# Autodesk Inventor assembly: CycloidalGearBoxV3_Assembly
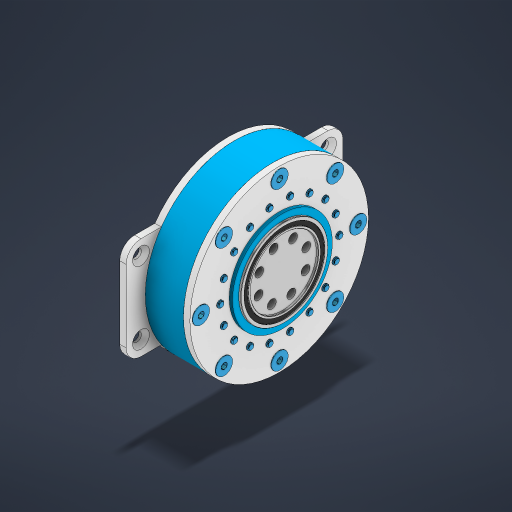
[picture p0: Inventor's stored thumbnail of the model, 512x512]
Saved by Autodesk Inventor 2024 (Build 280153000, 153)
## iProperties
Created: 2024-03-23
Part Number: CycloidalGearBoxV3_Assembly
Document SubType Name: Assembly
Designer: avsar
Author: avsar
## Documents named in this file (21)
- C:\Users\avsar\Documents\Inventor\RCR_Arm\Arm_V4\CycloidalGearBoxes\CycloidalGearboxV3\CycloidalGearBoxV3_Assembly.iam
- C:\Users\avsar\Documents\Inventor\RCR_Arm\Arm_V4\CycloidalGearBoxes\StageOneGearBox\HousingFaceInput.ipt
- C:\Users\avsar\Documents\Inventor\RCR_Arm\COTS\ISO Standard Hardware\Screws\Sockethead Screws\Countersunk Screws\M3 x 0.5mm\(M3 x 0.5 x 25) Sockethead Countersunk Screw.ipt
- C:\Users\avsar\Documents\Inventor\RCR_Arm\COTS\Motion\Bearings\Flanged Bearings\10x15x4mm Flanged Bearing.ipt
- C:\Users\avsar\Documents\Inventor\RCR_Arm\COTS\Motion\Bearings\Thrust Bearings\3mm ID x 8mm OD Thrust Ball Bearing.ipt
- C:\Users\avsar\Documents\Inventor\RCR_Arm\Arm_V4\CycloidalGearBoxes\CycloidalGearboxV3\RollerSpacers\ThrustRollerSpacer.ipt
- C:\Users\avsar\Documents\Inventor\RCR_Arm\Arm_V4\CycloidalGearBoxes\CycloidalGearboxV3\EccentricShaftSpacer.ipt
- C:\Users\avsar\Documents\Inventor\RCR_Arm\Arm_V4\CycloidalGearBoxes\CycloidalGearboxV3\CycloidalDisk.ipt
- C:\Users\avsar\Documents\Inventor\RCR_Arm\Arm_V4\CycloidalGearBoxes\CycloidalGearboxV3\EccentricShaft.ipt
- C:\Users\avsar\Documents\Inventor\RCR_Arm\COTS\Motion\Bearings\Standard Bearings\16mm ID x 22mm OD x 4mm Thickness Ball Bearing.ipt
- C:\Users\avsar\Documents\Inventor\RCR_Arm\COTS\ISO Standard Hardware\Screws\Sockethead Screws\Buttonhead Screws\M3 x 0.5mm\(M3 x 0.5 x 16) Sockethead Buttonhead Screw.ipt
- C:\Users\avsar\Documents\Inventor\RCR_Arm\Arm_V4\CycloidalGearBoxes\CycloidalGearboxV3\InnerBearingButtonheadShims.ipt
- C:\Users\avsar\Documents\Inventor\RCR_Arm\Arm_V4\CycloidalGearBoxes\CycloidalGearboxV3\InnerPins\InnerPinOutputSpacer.ipt
- C:\Users\avsar\Documents\Inventor\RCR_Arm\Arm_V4\CycloidalGearBoxes\CycloidalGearboxV3\OutPutPlate.ipt
- C:\Users\avsar\Documents\Inventor\RCR_Arm\Arm_V4\CycloidalGearBoxes\CycloidalGearboxV3\RollerSpacers\3mm ID x 4mm OD x 2mm Length Spacer.ipt
- C:\Users\avsar\Documents\Inventor\RCR_Arm\Arm_V4\CycloidalGearBoxes\CycloidalGearboxV3\RollerSpacers\StandardRollerSpacer.ipt
- C:\Users\avsar\Documents\Inventor\RCR_Arm\Arm_V4\CycloidalGearBoxes\CycloidalGearboxV3\HousingLid.ipt
- C:\Users\avsar\Documents\Inventor\RCR_Arm\Arm_V4\CycloidalGearBoxes\CycloidalGearboxV3\Gearbox_MainBody.ipt
- C:\Users\avsar\Documents\Inventor\RCR_Arm\COTS\goBilda\Motion\Bearings\32mm ID Flanged Ball Bearing (39mm OD, 5mm Thickness).ipt
- C:\Users\avsar\Documents\Inventor\RCR_Arm\Arm_V4\CycloidalGearBoxes\CycloidalGearboxV3\OutputBearingDistanceRing.ipt
- C:\Users\avsar\Documents\Inventor\RCR_Arm\COTS\ISO Standard Hardware\Screws\Sockethead Screws\Countersunk Screws\M4 x 0.7mm\(M4 x 0.7 x 10) Sockethead Countersunk Screw.ipt
## Components (107 placed, 20 different names)
1. HousingFaceInput:1 — Mate:1, Mate:2, Flush:1, Mate:3, Flush:2, Mate:4, Flush:3, Mate:5, Flush:4, Mate:6, Flush:5, Mate:7, Flush:6, Mate:8, Flush:7, Mate:9, Flush:8, Mate:10, Flush:9, Mate:11, Flush:10, Mate:12, Flush:11, Mate:13, Flush:12, Mate:14, Flush:13, Flush:14, Mate:15, Mate:16, Flush:15, Mate:17, Flush:16, Mate:18, Flush:17, Mate:19, Mate:20, Mate:21, Mate:26, Mate:91, Mate:97, Mate:103, Mate:109, Mate:115, Mate:129, Mate:131, Mate:133, Mate:135, Mate:137, Mate:139, Mate:141, Mate:143, Mate:145, Mate:147, Mate:149, Mate:151, Mate:154, Mate:155, Mate:156, Flush:20, Mate:163, Flush:21, Mate:164, Flush:22, Mate:165, Flush:23, Mate:166, Flush:24, Mate:167, Flush:25, Mate:168, Flush:26, Mate:169, Flush:27, Mate:170
2. 10x15x4mm Flanged Bearing:1 — Mate:20, Mate:21, Mate:30, Mate:31
3. EccentricShaftSpacer:1 — Mate:30, Mate:31, Mate:32, Mate:33
4. CycloidalDisk:1 — Flush:18, Mate:34, Mate:46, Tangent:1, Mate:51, Tangent:3, Mate:56, Tangent:5, Mate:69, Tangent:7, Mate:70, Tangent:9, Mate:71, Tangent:11, Tangent:13
5. EccentricShaft:1 — Mate:32, Mate:33, Mate:35, Mate:36, Mate:38, Mate:39
6. 16mm ID x 22mm OD x 4mm Thickness Ball Bearing:1 — Flush:18, Mate:34, Mate:35, Mate:36
7. CycloidalDisk:2 — Tangent:2, Tangent:4, Tangent:6, Tangent:8, Tangent:10, Tangent:12
8. OutPutPlate:1 — Mate:84, Mate:85, Mate:86
9. 16mm ID x 22mm OD x 4mm Thickness Ball Bearing:2 — Mate:38, Mate:39
10. StandardRollerSpacer:1 — Mate:129, Mate:130
11. StandardRollerSpacer:2 — Mate:131, Mate:132
12. StandardRollerSpacer:3 — Mate:133, Mate:134
13. StandardRollerSpacer:4 — Mate:135, Mate:136, Mate:153
14. StandardRollerSpacer:5 — Mate:137, Mate:138
15. StandardRollerSpacer:6 — Mate:139, Mate:140
16. StandardRollerSpacer:7 — Mate:141, Mate:142
17. StandardRollerSpacer:8 — Mate:143, Mate:144
18. StandardRollerSpacer:9 — Mate:145, Mate:146
19. StandardRollerSpacer:10 — Mate:147, Mate:148
20. StandardRollerSpacer:11 — Mate:149, Mate:150
21. StandardRollerSpacer:12 — Mate:151, Mate:152
22. HousingLid:1 — Mate:153, Mate:157, Mate:158, Mate:161, Mate:162, Flush:28, Mate:171, Flush:29, Mate:172, Flush:30, Mate:173, Flush:31, Mate:174, Flush:32, Mate:175, Flush:33, Mate:176, Flush:34, Mate:177, Flush:35, Mate:178
23. Gearbox_MainBody:1 — Mate:154, Mate:155, Mate:156, Mate:157, Mate:158
24. 32mm ID Flanged Ball Bearing (39mm OD, 5mm Thickness):1 — Mate:159, Mate:160, Mate:162
25. OutputBearingDistanceRing:1 — Mate:159, Mate:160, Mate:161
26. (M4 x 0.7 x 10) Sockethead Countersunk Screw:1 — Flush:20, Mate:163
27. (M4 x 0.7 x 10) Sockethead Countersunk Screw:2 — Flush:21, Mate:164
28. (M4 x 0.7 x 10) Sockethead Countersunk Screw:3 — Flush:22, Mate:165
29. (M4 x 0.7 x 10) Sockethead Countersunk Screw:4 — Flush:23, Mate:166
30. (M4 x 0.7 x 10) Sockethead Countersunk Screw:5 — Flush:24, Mate:167
31. (M4 x 0.7 x 10) Sockethead Countersunk Screw:6 — Flush:25, Mate:168
32. (M4 x 0.7 x 10) Sockethead Countersunk Screw:7 — Flush:26, Mate:169
33. (M4 x 0.7 x 10) Sockethead Countersunk Screw:8 — Flush:27, Mate:170
34. (M4 x 0.7 x 10) Sockethead Countersunk Screw:9 — Flush:28, Mate:171
35. (M4 x 0.7 x 10) Sockethead Countersunk Screw:10 — Flush:29, Mate:172
36. (M4 x 0.7 x 10) Sockethead Countersunk Screw:11 — Flush:30, Mate:173
37. (M4 x 0.7 x 10) Sockethead Countersunk Screw:12 — Flush:31, Mate:174
38. (M4 x 0.7 x 10) Sockethead Countersunk Screw:13 — Flush:32, Mate:175
39. (M4 x 0.7 x 10) Sockethead Countersunk Screw:14 — Flush:33, Mate:176
40. (M4 x 0.7 x 10) Sockethead Countersunk Screw:15 — Flush:34, Mate:177
41. (M4 x 0.7 x 10) Sockethead Countersunk Screw:16 — Flush:35, Mate:178
42. (M3 x 0.5 x 25) Sockethead Countersunk Screw:12 — Flush:11, Mate:13, Mate:98, Mate:126
43. (M3 x 0.5 x 25) Sockethead Countersunk Screw:13 — Flush:12, Mate:14, Mate:140
44. (M3 x 0.5 x 25) Sockethead Countersunk Screw:14 — Flush:13, Mate:15, Mate:138
45. (M3 x 0.5 x 25) Sockethead Countersunk Screw:15 — Flush:14, Mate:16, Mate:92, Mate:128
46. (M3 x 0.5 x 25) Sockethead Countersunk Screw:16 — Flush:15, Mate:17, Mate:136
47. (M3 x 0.5 x 25) Sockethead Countersunk Screw:17 — Flush:16, Mate:18, Mate:134
48. (M3 x 0.5 x 25) Sockethead Countersunk Screw:18 — Flush:17, Mate:19, Mate:25, Mate:28
49. (M3 x 0.5 x 25) Sockethead Countersunk Screw:1 — Mate:1, Mate:2, Mate:130
50. (M3 x 0.5 x 25) Sockethead Countersunk Screw:2 — Flush:1, Mate:3, Mate:132
51. (M3 x 0.5 x 25) Sockethead Countersunk Screw:3 — Flush:2, Mate:4, Mate:116, Mate:120
52. (M3 x 0.5 x 25) Sockethead Countersunk Screw:4 — Flush:3, Mate:5, Mate:152
53. (M3 x 0.5 x 25) Sockethead Countersunk Screw:5 — Flush:4, Mate:6, Mate:150
54. (M3 x 0.5 x 25) Sockethead Countersunk Screw:6 — Flush:5, Mate:7, Mate:110, Mate:122
55. (M3 x 0.5 x 25) Sockethead Countersunk Screw:7 — Flush:6, Mate:8, Mate:148
56. (M3 x 0.5 x 25) Sockethead Countersunk Screw:8 — Flush:7, Mate:9, Mate:146
57. (M3 x 0.5 x 25) Sockethead Countersunk Screw:9 — Flush:8, Mate:10, Mate:104, Mate:124
58. (M3 x 0.5 x 25) Sockethead Countersunk Screw:10 — Flush:9, Mate:11, Mate:144
59. (M3 x 0.5 x 25) Sockethead Countersunk Screw:11 — Flush:10, Mate:12, Mate:142
60. (M3 x 0.5 x 16) Sockethead Buttonhead Screw:1 — Mate:42, Mate:43, Mate:79
61. InnerBearingButtonheadShims:1 — Mate:42, Mate:43, Mate:44, Mate:45, Mate:46
62. ThrustRollerSpacer:2 — Mate:44, Mate:45, Tangent:1, Tangent:2, Mate:78
63. (M3 x 0.5 x 16) Sockethead Buttonhead Screw:2 — Mate:77
64. InnerBearingButtonheadShims:2 — Mate:51
65. ThrustRollerSpacer:3 — Tangent:3, Tangent:4, Mate:76
66. (M3 x 0.5 x 16) Sockethead Buttonhead Screw:3 — Mate:81, Mate:86
67. InnerBearingButtonheadShims:3 — Mate:56
68. ThrustRollerSpacer:4 — Tangent:5, Tangent:6, Mate:80
69. (M3 x 0.5 x 16) Sockethead Buttonhead Screw:4 — Mate:83
70. InnerBearingButtonheadShims:4 — Mate:69
71. ThrustRollerSpacer:5 — Tangent:7, Tangent:8, Mate:82
72. (M3 x 0.5 x 16) Sockethead Buttonhead Screw:5 — Mate:73
73. InnerBearingButtonheadShims:5 — Mate:70
74. ThrustRollerSpacer:6 — Tangent:9, Tangent:10, Mate:72
75. (M3 x 0.5 x 16) Sockethead Buttonhead Screw:6 — Mate:75, Mate:85
76. InnerBearingButtonheadShims:6 — Mate:71
77. ThrustRollerSpacer:7 — Tangent:11, Tangent:12, Mate:74
78. InnerPinOutputSpacer:1 — Mate:72, Mate:73
79. InnerPinOutputSpacer:2 — Mate:74, Mate:75, Mate:84
80. InnerPinOutputSpacer:3 — Mate:76, Mate:77
81. InnerPinOutputSpacer:4 — Mate:78, Mate:79
82. InnerPinOutputSpacer:5 — Mate:80, Mate:81
83. InnerPinOutputSpacer:6 — Mate:82, Mate:83
84. 3mm ID x 8mm OD Thrust Ball Bearing:5 — Mate:125
85. 3mm ID x 8mm OD Thrust Ball Bearing:6 — Mate:97
86. ThrustRollerSpacer:9 — Mate:98
87. 3mm ID x 8mm OD Thrust Ball Bearing:7 — Mate:123
88. 3mm ID x 8mm OD Thrust Ball Bearing:8 — Mate:103
89. ThrustRollerSpacer:10 — Mate:104
90. 3mm ID x 8mm OD Thrust Ball Bearing:9 — Mate:121
91. 3mm ID x 8mm OD Thrust Ball Bearing:10 — Mate:109
92. ThrustRollerSpacer:11 — Mate:110
93. 3mm ID x 8mm OD Thrust Ball Bearing:11 — Mate:119
94. 3mm ID x 8mm OD Thrust Ball Bearing:12 — Mate:115
95. ThrustRollerSpacer:12 — Mate:116
96. 3mm ID x 4mm OD x 2mm Length Spacer:1 — Mate:117, Mate:118
97. 3mm ID x 4mm OD x 2mm Length Spacer:2 — Mate:123, Mate:124
98. 3mm ID x 4mm OD x 2mm Length Spacer:3 — Mate:125, Mate:126
99. 3mm ID x 4mm OD x 2mm Length Spacer:4 — Mate:127, Mate:128
100. 3mm ID x 4mm OD x 2mm Length Spacer:5 — Mate:121, Mate:122
101. 3mm ID x 4mm OD x 2mm Length Spacer:6 — Mate:119, Mate:120
102. 3mm ID x 8mm OD Thrust Ball Bearing:3 — Mate:127
103. 3mm ID x 8mm OD Thrust Ball Bearing:4 — Mate:91
104. ThrustRollerSpacer:8 — Mate:92
105. 3mm ID x 8mm OD Thrust Ball Bearing:1 — Mate:25, Mate:26, Mate:27, Mate:29
106. 3mm ID x 8mm OD Thrust Ball Bearing:2 — Mate:40, Mate:41, Mate:117
107. ThrustRollerSpacer:1 — Mate:27, Mate:28, Mate:29, Mate:40, Mate:41, Tangent:13, Mate:118
## Relationships (223: Mate 175, Flush 35, Tangent 13)
- Mate:1: HousingFaceInput:1 ↔ (M3 x 0.5 x 25) Sockethead Countersunk Screw:1
- Mate:2: HousingFaceInput:1 ↔ (M3 x 0.5 x 25) Sockethead Countersunk Screw:1
- Flush:1 (-0.085 mm): HousingFaceInput:1 ↔ (M3 x 0.5 x 25) Sockethead Countersunk Screw:2
- Mate:3: HousingFaceInput:1 ↔ (M3 x 0.5 x 25) Sockethead Countersunk Screw:2
- Flush:2 (-0.085 mm): HousingFaceInput:1 ↔ (M3 x 0.5 x 25) Sockethead Countersunk Screw:3
- Mate:4: HousingFaceInput:1 ↔ (M3 x 0.5 x 25) Sockethead Countersunk Screw:3
- Flush:3 (-0.085 mm): HousingFaceInput:1 ↔ (M3 x 0.5 x 25) Sockethead Countersunk Screw:4
- Mate:5: HousingFaceInput:1 ↔ (M3 x 0.5 x 25) Sockethead Countersunk Screw:4
- Flush:4 (-0.085 mm): HousingFaceInput:1 ↔ (M3 x 0.5 x 25) Sockethead Countersunk Screw:5
- Mate:6: HousingFaceInput:1 ↔ (M3 x 0.5 x 25) Sockethead Countersunk Screw:5
- Flush:5 (-0.085 mm): HousingFaceInput:1 ↔ (M3 x 0.5 x 25) Sockethead Countersunk Screw:6
- Mate:7: HousingFaceInput:1 ↔ (M3 x 0.5 x 25) Sockethead Countersunk Screw:6
- Flush:6 (-0.085 mm): HousingFaceInput:1 ↔ (M3 x 0.5 x 25) Sockethead Countersunk Screw:7
- Mate:8: HousingFaceInput:1 ↔ (M3 x 0.5 x 25) Sockethead Countersunk Screw:7
- Flush:7 (-0.085 mm): HousingFaceInput:1 ↔ (M3 x 0.5 x 25) Sockethead Countersunk Screw:8
- Mate:9: HousingFaceInput:1 ↔ (M3 x 0.5 x 25) Sockethead Countersunk Screw:8
- Flush:8 (-0.085 mm): HousingFaceInput:1 ↔ (M3 x 0.5 x 25) Sockethead Countersunk Screw:9
- Mate:10: HousingFaceInput:1 ↔ (M3 x 0.5 x 25) Sockethead Countersunk Screw:9
- Flush:9 (-0.085 mm): HousingFaceInput:1 ↔ (M3 x 0.5 x 25) Sockethead Countersunk Screw:10
- Mate:11: HousingFaceInput:1 ↔ (M3 x 0.5 x 25) Sockethead Countersunk Screw:10
- Flush:10 (-0.085 mm): HousingFaceInput:1 ↔ (M3 x 0.5 x 25) Sockethead Countersunk Screw:11
- Mate:12: HousingFaceInput:1 ↔ (M3 x 0.5 x 25) Sockethead Countersunk Screw:11
- Flush:11 (-0.085 mm): HousingFaceInput:1 ↔ (M3 x 0.5 x 25) Sockethead Countersunk Screw:12
- Mate:13: HousingFaceInput:1 ↔ (M3 x 0.5 x 25) Sockethead Countersunk Screw:12
- Flush:12 (-0.085 mm): HousingFaceInput:1 ↔ (M3 x 0.5 x 25) Sockethead Countersunk Screw:13
- Mate:14: HousingFaceInput:1 ↔ (M3 x 0.5 x 25) Sockethead Countersunk Screw:13
- Flush:13 (-0.085 mm): HousingFaceInput:1 ↔ (M3 x 0.5 x 25) Sockethead Countersunk Screw:14
- Flush:14 (-0.085 mm): HousingFaceInput:1 ↔ (M3 x 0.5 x 25) Sockethead Countersunk Screw:15
- Mate:15: HousingFaceInput:1 ↔ (M3 x 0.5 x 25) Sockethead Countersunk Screw:14
- Mate:16: HousingFaceInput:1 ↔ (M3 x 0.5 x 25) Sockethead Countersunk Screw:15
- Flush:15 (-0.085 mm): HousingFaceInput:1 ↔ (M3 x 0.5 x 25) Sockethead Countersunk Screw:16
- Mate:17: HousingFaceInput:1 ↔ (M3 x 0.5 x 25) Sockethead Countersunk Screw:16
- Flush:16 (-0.085 mm): HousingFaceInput:1 ↔ (M3 x 0.5 x 25) Sockethead Countersunk Screw:17
- Mate:18: HousingFaceInput:1 ↔ (M3 x 0.5 x 25) Sockethead Countersunk Screw:17
- Flush:17 (-0.085 mm): HousingFaceInput:1 ↔ (M3 x 0.5 x 25) Sockethead Countersunk Screw:18
- Mate:19: HousingFaceInput:1 ↔ (M3 x 0.5 x 25) Sockethead Countersunk Screw:18
- Mate:20: HousingFaceInput:1 ↔ 10x15x4mm Flanged Bearing:1
- Mate:21: HousingFaceInput:1 ↔ 10x15x4mm Flanged Bearing:1
- Mate:25: (M3 x 0.5 x 25) Sockethead Countersunk Screw:18 ↔ 3mm ID x 8mm OD Thrust Ball Bearing:1
- Mate:26: HousingFaceInput:1 ↔ 3mm ID x 8mm OD Thrust Ball Bearing:1
- Mate:27: 3mm ID x 8mm OD Thrust Ball Bearing:1 ↔ ThrustRollerSpacer:1
- Mate:28: (M3 x 0.5 x 25) Sockethead Countersunk Screw:18 ↔ ThrustRollerSpacer:1
- Mate:29: 3mm ID x 8mm OD Thrust Ball Bearing:1 ↔ ThrustRollerSpacer:1
- Mate:30: 10x15x4mm Flanged Bearing:1 ↔ EccentricShaftSpacer:1
- Mate:31: 10x15x4mm Flanged Bearing:1 ↔ EccentricShaftSpacer:1
- Mate:32: EccentricShaftSpacer:1 ↔ EccentricShaft:1
- Mate:33: EccentricShaftSpacer:1 ↔ EccentricShaft:1
- Flush:18: CycloidalDisk:1 ↔ 16mm ID x 22mm OD x 4mm Thickness Ball Bearing:1
- Mate:34: CycloidalDisk:1 ↔ 16mm ID x 22mm OD x 4mm Thickness Ball Bearing:1
- Mate:35: EccentricShaft:1 ↔ 16mm ID x 22mm OD x 4mm Thickness Ball Bearing:1
- Mate:36: EccentricShaft:1 ↔ 16mm ID x 22mm OD x 4mm Thickness Ball Bearing:1
- [Flush]: CycloidalDisk:2 ↔ 16mm ID x 22mm OD x 4mm Thickness Ball Bearing:2
- [Mate]: CycloidalDisk:2 ↔ 16mm ID x 22mm OD x 4mm Thickness Ball Bearing:2
- Mate:38: EccentricShaft:1 ↔ 16mm ID x 22mm OD x 4mm Thickness Ball Bearing:2
- Mate:39: EccentricShaft:1 ↔ 16mm ID x 22mm OD x 4mm Thickness Ball Bearing:2
- Mate:40: 3mm ID x 8mm OD Thrust Ball Bearing:2 ↔ ThrustRollerSpacer:1
- Mate:41: 3mm ID x 8mm OD Thrust Ball Bearing:2 ↔ ThrustRollerSpacer:1
- Mate:42: (M3 x 0.5 x 16) Sockethead Buttonhead Screw:1 ↔ InnerBearingButtonheadShims:1
- Mate:43: (M3 x 0.5 x 16) Sockethead Buttonhead Screw:1 ↔ InnerBearingButtonheadShims:1
- Mate:44: InnerBearingButtonheadShims:1 ↔ ThrustRollerSpacer:2
- Mate:45: InnerBearingButtonheadShims:1 ↔ ThrustRollerSpacer:2
- Mate:46: CycloidalDisk:1 ↔ InnerBearingButtonheadShims:1
- Tangent:1: CycloidalDisk:1 ↔ ThrustRollerSpacer:2
- Tangent:2: CycloidalDisk:2 ↔ ThrustRollerSpacer:2
- [Mate]: (M3 x 0.5 x 16) Sockethead Buttonhead Screw:2 ↔ InnerBearingButtonheadShims:2
- [Mate]: (M3 x 0.5 x 16) Sockethead Buttonhead Screw:2 ↔ InnerBearingButtonheadShims:2
- [Mate]: InnerBearingButtonheadShims:2 ↔ ThrustRollerSpacer:3
- [Mate]: InnerBearingButtonheadShims:2 ↔ ThrustRollerSpacer:3
- Mate:51: CycloidalDisk:1 ↔ InnerBearingButtonheadShims:2
- Tangent:3: CycloidalDisk:1 ↔ ThrustRollerSpacer:3
- Tangent:4: CycloidalDisk:2 ↔ ThrustRollerSpacer:3
- [Mate]: (M3 x 0.5 x 16) Sockethead Buttonhead Screw:3 ↔ InnerBearingButtonheadShims:3
- [Mate]: (M3 x 0.5 x 16) Sockethead Buttonhead Screw:3 ↔ InnerBearingButtonheadShims:3
- [Mate]: InnerBearingButtonheadShims:3 ↔ ThrustRollerSpacer:4
- [Mate]: InnerBearingButtonheadShims:3 ↔ ThrustRollerSpacer:4
- Mate:56: CycloidalDisk:1 ↔ InnerBearingButtonheadShims:3
- Tangent:5: CycloidalDisk:1 ↔ ThrustRollerSpacer:4
- Tangent:6: CycloidalDisk:2 ↔ ThrustRollerSpacer:4
- [Mate]: (M3 x 0.5 x 16) Sockethead Buttonhead Screw:4 ↔ InnerBearingButtonheadShims:4
- [Mate]: (M3 x 0.5 x 16) Sockethead Buttonhead Screw:4 ↔ InnerBearingButtonheadShims:4
- [Mate]: InnerBearingButtonheadShims:4 ↔ ThrustRollerSpacer:5
- [Mate]: InnerBearingButtonheadShims:4 ↔ ThrustRollerSpacer:5
- [Mate]: (M3 x 0.5 x 16) Sockethead Buttonhead Screw:5 ↔ InnerBearingButtonheadShims:5
- [Mate]: (M3 x 0.5 x 16) Sockethead Buttonhead Screw:5 ↔ InnerBearingButtonheadShims:5
- [Mate]: InnerBearingButtonheadShims:5 ↔ ThrustRollerSpacer:6
- [Mate]: InnerBearingButtonheadShims:5 ↔ ThrustRollerSpacer:6
- [Mate]: (M3 x 0.5 x 16) Sockethead Buttonhead Screw:6 ↔ InnerBearingButtonheadShims:6
- [Mate]: (M3 x 0.5 x 16) Sockethead Buttonhead Screw:6 ↔ InnerBearingButtonheadShims:6
- [Mate]: InnerBearingButtonheadShims:6 ↔ ThrustRollerSpacer:7
- [Mate]: InnerBearingButtonheadShims:6 ↔ ThrustRollerSpacer:7
- Mate:69: CycloidalDisk:1 ↔ InnerBearingButtonheadShims:4
- Tangent:7: CycloidalDisk:1 ↔ ThrustRollerSpacer:5
- Tangent:8: CycloidalDisk:2 ↔ ThrustRollerSpacer:5
- Mate:70: CycloidalDisk:1 ↔ InnerBearingButtonheadShims:5
- Tangent:9: CycloidalDisk:1 ↔ ThrustRollerSpacer:6
- Tangent:10: CycloidalDisk:2 ↔ ThrustRollerSpacer:6
- Mate:71: CycloidalDisk:1 ↔ InnerBearingButtonheadShims:6
- Tangent:11: CycloidalDisk:1 ↔ ThrustRollerSpacer:7
- Tangent:12: CycloidalDisk:2 ↔ ThrustRollerSpacer:7
- Mate:72: ThrustRollerSpacer:6 ↔ InnerPinOutputSpacer:1
- Mate:73: (M3 x 0.5 x 16) Sockethead Buttonhead Screw:5 ↔ InnerPinOutputSpacer:1
- Mate:74: ThrustRollerSpacer:7 ↔ InnerPinOutputSpacer:2
- Mate:75: (M3 x 0.5 x 16) Sockethead Buttonhead Screw:6 ↔ InnerPinOutputSpacer:2
- Mate:76: ThrustRollerSpacer:3 ↔ InnerPinOutputSpacer:3
- Mate:77: (M3 x 0.5 x 16) Sockethead Buttonhead Screw:2 ↔ InnerPinOutputSpacer:3
- Mate:78: ThrustRollerSpacer:2 ↔ InnerPinOutputSpacer:4
- Mate:79: (M3 x 0.5 x 16) Sockethead Buttonhead Screw:1 ↔ InnerPinOutputSpacer:4
- Mate:80: ThrustRollerSpacer:4 ↔ InnerPinOutputSpacer:5
- Mate:81: (M3 x 0.5 x 16) Sockethead Buttonhead Screw:3 ↔ InnerPinOutputSpacer:5
- Mate:82: ThrustRollerSpacer:5 ↔ InnerPinOutputSpacer:6
- Mate:83: (M3 x 0.5 x 16) Sockethead Buttonhead Screw:4 ↔ InnerPinOutputSpacer:6
- Mate:84: OutPutPlate:1 ↔ InnerPinOutputSpacer:2
- Mate:85: OutPutPlate:1 ↔ (M3 x 0.5 x 16) Sockethead Buttonhead Screw:6
- Mate:86: OutPutPlate:1 ↔ (M3 x 0.5 x 16) Sockethead Buttonhead Screw:3
- Tangent:13: CycloidalDisk:1 ↔ ThrustRollerSpacer:1
- [Mate]: 3mm ID x 8mm OD Thrust Ball Bearing:3 ↔ ThrustRollerSpacer:8
- [Mate]: 3mm ID x 8mm OD Thrust Ball Bearing:3 ↔ ThrustRollerSpacer:8
- [Mate]: 3mm ID x 8mm OD Thrust Ball Bearing:4 ↔ ThrustRollerSpacer:8
- [Mate]: 3mm ID x 8mm OD Thrust Ball Bearing:4 ↔ ThrustRollerSpacer:8
- Mate:91: HousingFaceInput:1 ↔ 3mm ID x 8mm OD Thrust Ball Bearing:4
- Mate:92: (M3 x 0.5 x 25) Sockethead Countersunk Screw:15 ↔ ThrustRollerSpacer:8
- [Mate]: 3mm ID x 8mm OD Thrust Ball Bearing:5 ↔ ThrustRollerSpacer:9
- [Mate]: 3mm ID x 8mm OD Thrust Ball Bearing:5 ↔ ThrustRollerSpacer:9
- [Mate]: 3mm ID x 8mm OD Thrust Ball Bearing:6 ↔ ThrustRollerSpacer:9
- [Mate]: 3mm ID x 8mm OD Thrust Ball Bearing:6 ↔ ThrustRollerSpacer:9
- Mate:97: HousingFaceInput:1 ↔ 3mm ID x 8mm OD Thrust Ball Bearing:6
- Mate:98: (M3 x 0.5 x 25) Sockethead Countersunk Screw:12 ↔ ThrustRollerSpacer:9
- [Mate]: 3mm ID x 8mm OD Thrust Ball Bearing:7 ↔ ThrustRollerSpacer:10
- [Mate]: 3mm ID x 8mm OD Thrust Ball Bearing:7 ↔ ThrustRollerSpacer:10
- [Mate]: 3mm ID x 8mm OD Thrust Ball Bearing:8 ↔ ThrustRollerSpacer:10
- [Mate]: 3mm ID x 8mm OD Thrust Ball Bearing:8 ↔ ThrustRollerSpacer:10
- Mate:103: HousingFaceInput:1 ↔ 3mm ID x 8mm OD Thrust Ball Bearing:8
- Mate:104: (M3 x 0.5 x 25) Sockethead Countersunk Screw:9 ↔ ThrustRollerSpacer:10
- [Mate]: 3mm ID x 8mm OD Thrust Ball Bearing:9 ↔ ThrustRollerSpacer:11
- [Mate]: 3mm ID x 8mm OD Thrust Ball Bearing:9 ↔ ThrustRollerSpacer:11
- [Mate]: 3mm ID x 8mm OD Thrust Ball Bearing:10 ↔ ThrustRollerSpacer:11
- [Mate]: 3mm ID x 8mm OD Thrust Ball Bearing:10 ↔ ThrustRollerSpacer:11
- Mate:109: HousingFaceInput:1 ↔ 3mm ID x 8mm OD Thrust Ball Bearing:10
- Mate:110: (M3 x 0.5 x 25) Sockethead Countersunk Screw:6 ↔ ThrustRollerSpacer:11
- [Mate]: 3mm ID x 8mm OD Thrust Ball Bearing:11 ↔ ThrustRollerSpacer:12
- [Mate]: 3mm ID x 8mm OD Thrust Ball Bearing:11 ↔ ThrustRollerSpacer:12
- [Mate]: 3mm ID x 8mm OD Thrust Ball Bearing:12 ↔ ThrustRollerSpacer:12
- [Mate]: 3mm ID x 8mm OD Thrust Ball Bearing:12 ↔ ThrustRollerSpacer:12
- Mate:115: HousingFaceInput:1 ↔ 3mm ID x 8mm OD Thrust Ball Bearing:12
- Mate:116: (M3 x 0.5 x 25) Sockethead Countersunk Screw:3 ↔ ThrustRollerSpacer:12
- Mate:117: 3mm ID x 4mm OD x 2mm Length Spacer:1 ↔ 3mm ID x 8mm OD Thrust Ball Bearing:2
- Mate:118: 3mm ID x 4mm OD x 2mm Length Spacer:1 ↔ ThrustRollerSpacer:1
- Mate:119: 3mm ID x 8mm OD Thrust Ball Bearing:11 ↔ 3mm ID x 4mm OD x 2mm Length Spacer:6
- Mate:120: (M3 x 0.5 x 25) Sockethead Countersunk Screw:3 ↔ 3mm ID x 4mm OD x 2mm Length Spacer:6
- Mate:121: 3mm ID x 8mm OD Thrust Ball Bearing:9 ↔ 3mm ID x 4mm OD x 2mm Length Spacer:5
- Mate:122: (M3 x 0.5 x 25) Sockethead Countersunk Screw:6 ↔ 3mm ID x 4mm OD x 2mm Length Spacer:5
- Mate:123: 3mm ID x 8mm OD Thrust Ball Bearing:7 ↔ 3mm ID x 4mm OD x 2mm Length Spacer:2
- Mate:124: (M3 x 0.5 x 25) Sockethead Countersunk Screw:9 ↔ 3mm ID x 4mm OD x 2mm Length Spacer:2
- Mate:125: 3mm ID x 8mm OD Thrust Ball Bearing:5 ↔ 3mm ID x 4mm OD x 2mm Length Spacer:3
- Mate:126: (M3 x 0.5 x 25) Sockethead Countersunk Screw:12 ↔ 3mm ID x 4mm OD x 2mm Length Spacer:3
- Mate:127: 3mm ID x 4mm OD x 2mm Length Spacer:4 ↔ 3mm ID x 8mm OD Thrust Ball Bearing:3
- Mate:128: (M3 x 0.5 x 25) Sockethead Countersunk Screw:15 ↔ 3mm ID x 4mm OD x 2mm Length Spacer:4
- Mate:129: HousingFaceInput:1 ↔ StandardRollerSpacer:1
- Mate:130: StandardRollerSpacer:1 ↔ (M3 x 0.5 x 25) Sockethead Countersunk Screw:1
- Mate:131: HousingFaceInput:1 ↔ StandardRollerSpacer:2
- Mate:132: StandardRollerSpacer:2 ↔ (M3 x 0.5 x 25) Sockethead Countersunk Screw:2
- Mate:133: HousingFaceInput:1 ↔ StandardRollerSpacer:3
- Mate:134: StandardRollerSpacer:3 ↔ (M3 x 0.5 x 25) Sockethead Countersunk Screw:17
- Mate:135: HousingFaceInput:1 ↔ StandardRollerSpacer:4
- Mate:136: StandardRollerSpacer:4 ↔ (M3 x 0.5 x 25) Sockethead Countersunk Screw:16
- Mate:137: HousingFaceInput:1 ↔ StandardRollerSpacer:5
- Mate:138: StandardRollerSpacer:5 ↔ (M3 x 0.5 x 25) Sockethead Countersunk Screw:14
- Mate:139: HousingFaceInput:1 ↔ StandardRollerSpacer:6
- Mate:140: StandardRollerSpacer:6 ↔ (M3 x 0.5 x 25) Sockethead Countersunk Screw:13
- Mate:141: HousingFaceInput:1 ↔ StandardRollerSpacer:7
- Mate:142: StandardRollerSpacer:7 ↔ (M3 x 0.5 x 25) Sockethead Countersunk Screw:11
- Mate:143: HousingFaceInput:1 ↔ StandardRollerSpacer:8
- Mate:144: StandardRollerSpacer:8 ↔ (M3 x 0.5 x 25) Sockethead Countersunk Screw:10
- Mate:145: HousingFaceInput:1 ↔ StandardRollerSpacer:9
- Mate:146: StandardRollerSpacer:9 ↔ (M3 x 0.5 x 25) Sockethead Countersunk Screw:8
- Mate:147: HousingFaceInput:1 ↔ StandardRollerSpacer:10
- Mate:148: StandardRollerSpacer:10 ↔ (M3 x 0.5 x 25) Sockethead Countersunk Screw:7
- Mate:149: HousingFaceInput:1 ↔ StandardRollerSpacer:11
- Mate:150: StandardRollerSpacer:11 ↔ (M3 x 0.5 x 25) Sockethead Countersunk Screw:5
- Mate:151: HousingFaceInput:1 ↔ StandardRollerSpacer:12
- Mate:152: StandardRollerSpacer:12 ↔ (M3 x 0.5 x 25) Sockethead Countersunk Screw:4
- Mate:153: StandardRollerSpacer:4 ↔ HousingLid:1
- Mate:154: HousingFaceInput:1 ↔ Gearbox_MainBody:1
- Mate:155: HousingFaceInput:1 ↔ Gearbox_MainBody:1
- Mate:156: HousingFaceInput:1 ↔ Gearbox_MainBody:1
- Mate:157: HousingLid:1 ↔ Gearbox_MainBody:1
- Mate:158: HousingLid:1 ↔ Gearbox_MainBody:1
- Mate:159: 32mm ID Flanged Ball Bearing (39mm OD, 5mm Thickness):1 ↔ OutputBearingDistanceRing:1
- Mate:160: 32mm ID Flanged Ball Bearing (39mm OD, 5mm Thickness):1 ↔ OutputBearingDistanceRing:1
- Mate:161: HousingLid:1 ↔ OutputBearingDistanceRing:1
- Mate:162: HousingLid:1 ↔ 32mm ID Flanged Ball Bearing (39mm OD, 5mm Thickness):1
- Flush:20 (-0.3 mm): HousingFaceInput:1 ↔ (M4 x 0.7 x 10) Sockethead Countersunk Screw:1
- Mate:163: HousingFaceInput:1 ↔ (M4 x 0.7 x 10) Sockethead Countersunk Screw:1
- Flush:21 (-0.3 mm): HousingFaceInput:1 ↔ (M4 x 0.7 x 10) Sockethead Countersunk Screw:2
- Mate:164: HousingFaceInput:1 ↔ (M4 x 0.7 x 10) Sockethead Countersunk Screw:2
- Flush:22 (-0.3 mm): HousingFaceInput:1 ↔ (M4 x 0.7 x 10) Sockethead Countersunk Screw:3
- Mate:165: HousingFaceInput:1 ↔ (M4 x 0.7 x 10) Sockethead Countersunk Screw:3
- Flush:23 (-0.3 mm): HousingFaceInput:1 ↔ (M4 x 0.7 x 10) Sockethead Countersunk Screw:4
- Mate:166: HousingFaceInput:1 ↔ (M4 x 0.7 x 10) Sockethead Countersunk Screw:4
- Flush:24 (-0.3 mm): HousingFaceInput:1 ↔ (M4 x 0.7 x 10) Sockethead Countersunk Screw:5
- Mate:167: HousingFaceInput:1 ↔ (M4 x 0.7 x 10) Sockethead Countersunk Screw:5
- Flush:25 (-0.3 mm): HousingFaceInput:1 ↔ (M4 x 0.7 x 10) Sockethead Countersunk Screw:6
- Mate:168: HousingFaceInput:1 ↔ (M4 x 0.7 x 10) Sockethead Countersunk Screw:6
- Flush:26 (-0.3 mm): HousingFaceInput:1 ↔ (M4 x 0.7 x 10) Sockethead Countersunk Screw:7
- Mate:169: HousingFaceInput:1 ↔ (M4 x 0.7 x 10) Sockethead Countersunk Screw:7
- Flush:27 (-0.3 mm): HousingFaceInput:1 ↔ (M4 x 0.7 x 10) Sockethead Countersunk Screw:8
- Mate:170: HousingFaceInput:1 ↔ (M4 x 0.7 x 10) Sockethead Countersunk Screw:8
- Flush:28 (-0.3 mm): HousingLid:1 ↔ (M4 x 0.7 x 10) Sockethead Countersunk Screw:9
- Mate:171: HousingLid:1 ↔ (M4 x 0.7 x 10) Sockethead Countersunk Screw:9
- Flush:29 (-0.3 mm): HousingLid:1 ↔ (M4 x 0.7 x 10) Sockethead Countersunk Screw:10
- Mate:172: HousingLid:1 ↔ (M4 x 0.7 x 10) Sockethead Countersunk Screw:10
- Flush:30 (-0.3 mm): HousingLid:1 ↔ (M4 x 0.7 x 10) Sockethead Countersunk Screw:11
- Mate:173: HousingLid:1 ↔ (M4 x 0.7 x 10) Sockethead Countersunk Screw:11
- Flush:31 (-0.3 mm): HousingLid:1 ↔ (M4 x 0.7 x 10) Sockethead Countersunk Screw:12
- Mate:174: HousingLid:1 ↔ (M4 x 0.7 x 10) Sockethead Countersunk Screw:12
- Flush:32 (-0.3 mm): HousingLid:1 ↔ (M4 x 0.7 x 10) Sockethead Countersunk Screw:13
- Mate:175: HousingLid:1 ↔ (M4 x 0.7 x 10) Sockethead Countersunk Screw:13
- Flush:33 (-0.3 mm): HousingLid:1 ↔ (M4 x 0.7 x 10) Sockethead Countersunk Screw:14
- Mate:176: HousingLid:1 ↔ (M4 x 0.7 x 10) Sockethead Countersunk Screw:14
- Flush:34 (-0.3 mm): HousingLid:1 ↔ (M4 x 0.7 x 10) Sockethead Countersunk Screw:15
- Mate:177: HousingLid:1 ↔ (M4 x 0.7 x 10) Sockethead Countersunk Screw:15
- Flush:35 (-0.3 mm): HousingLid:1 ↔ (M4 x 0.7 x 10) Sockethead Countersunk Screw:16
- Mate:178: HousingLid:1 ↔ (M4 x 0.7 x 10) Sockethead Countersunk Screw:16
## Named parameters: d60_d54 = 0 mm, d61_d55 = 0 mm, d83_d67 = 0 mm, d84_d68 = 0 mm, d85_d78 = 0 mm, d86_d79 = 0 mm, d90_d67 = 0 mm, d91_d68 = 0 mm, d92_d78 = 0 mm, d93_d79 = 0 mm, d97_d67 = 0 mm, d98_d68 = 0 mm, d99_d78 = 0 mm, d100_d79 = 0 mm, d101_d67 = 0 mm, d102_d68 = 0 mm, d103_d78 = 0 mm, d104_d79 = 0 mm, d105_d67 = 0 mm, d106_d68 = 0 mm, d107_d78 = 0 mm, d108_d79 = 0 mm, d138_d64 = 0 mm, d139_d65 = 0 mm, d140_d47 = 0 mm, d141_d49 = 0 mm, d144_d64 = 0 mm, d145_d65 = 0 mm, d146_d47 = 0 mm, d147_d49 = 0 mm, d150_d64 = 0 mm, d151_d65 = 0 mm, d152_d47 = 0 mm, d153_d49 = 0 mm, d156_d64 = 0 mm, d157_d65 = 0 mm, d158_d47 = 0 mm, d159_d49 = 0 mm, d162_d64 = 0 mm, d163_d65 = 0 mm, d164_d47 = 0 mm, d165_d49 = 0 mm
